# Autodesk Inventor assembly: ASSEMBLY_Y_axis_motor
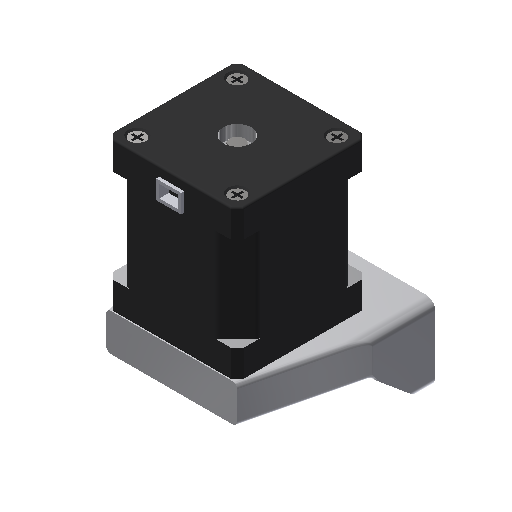
[picture p0: Inventor's stored thumbnail of the model, 512x512]
Saved by Autodesk Inventor 2026.1 (Build 301233000, 233)
## iProperties
Created: 2018-07-08
Part Number: ASSEMBLY_Y_axis_motor
Document SubType Name: Assembly
Designer: Andrzej
Author: Andrzej
## Documents named in this file (6)
- C:\Users\Andrzej\OneDrive\_DRIVE_SYNCH_FILES\__ BYTECHLAB PROJECTS\MLTDIS - SMD Parts Sorting Machine\MCAD\1_REV1\ASSEMBLY_XY_AXIS_REVA\ASSEMBLY_Y_axis_motor.iam
- C:\Users\Andrzej\OneDrive\_DRIVE_SYNCH_FILES\__ BYTECHLAB PROJECTS\MLTDIS - SMD Parts Sorting Machine\MCAD\1_REV1\ASSEMBLY_XY_AXIS_REVA\3DP_PLA_Nema_17_motor_mount.ipt
- C:\Users\Andrzej\OneDrive\_DRIVE_SYNCH_FILES\__ BYTECHLAB PROJECTS\MLTDIS - SMD Parts Sorting Machine\MCAD\1_REV1\__COTS_PARTS\COTS_GENERIC_NEMA_17_Stepper_motor.ipt
- C:\Users\Andrzej\OneDrive\_DRIVE_SYNCH_FILES\__ BYTECHLAB PROJECTS\MLTDIS - SMD Parts Sorting Machine\MCAD\1_REV1\__COTS_PARTS\COTS_GENERIC_GT2_20T_Pulley.ipt
- C:\Users\Andrzej\OneDrive\_DRIVE_SYNCH_FILES\__ BYTECHLAB PROJECTS\MLTDIS - SMD Parts Sorting Machine\MCAD\1_REV1\__CONTENT_CENTER_PARTS\en-US\DIN 125-2  A\DIN 125-2 - A 3,2A.ipt
- C:\Users\Andrzej\OneDrive\_DRIVE_SYNCH_FILES\__ BYTECHLAB PROJECTS\MLTDIS - SMD Parts Sorting Machine\MCAD\1_REV1\__CONTENT_CENTER_PARTS\en-US\ISO 7380-1\ISO 7380-1 - M3 x 20.ipt
## Components (11 placed, 5 different names)
1. 3DP_PLA_Nema_17_motor_mount:1 — Mate:1, Mate:2, Flush:1, Mate:4, Mate:5, Mate:6, Mate:7, Mate:8, Mate:9, Mate:10, Mate:11
2. COTS_GENERIC_NEMA_17_Stepper_motor:1 — Mate:1, Mate:2, Flush:1, Mate:3, Flush:2
3. COTS_GENERIC_GT2_20T_Pulley:1 — Mate:3, Flush:2
4. DIN 125-2 A A 3,2:1 — Mate:4, Mate:5, Insert:1
5. ISO 7380-1 M3 x 20:1 — Insert:1
6. DIN 125-2 A A 3,2:2 — Mate:6, Mate:7, Insert:2
7. DIN 125-2 A A 3,2:3 — Mate:8, Mate:9, Insert:3
8. DIN 125-2 A A 3,2:4 — Mate:10, Mate:11, Insert:4
9. ISO 7380-1 M3 x 20:2 — Insert:2
10. ISO 7380-1 M3 x 20:3 — Insert:3
11. ISO 7380-1 M3 x 20:4 — Insert:4
## Relationships (17: Mate 11, Insert 4, Flush 2)
- Mate:1: 3DP_PLA_Nema_17_motor_mount:1 ↔ COTS_GENERIC_NEMA_17_Stepper_motor:1
- Mate:2: 3DP_PLA_Nema_17_motor_mount:1 ↔ COTS_GENERIC_NEMA_17_Stepper_motor:1
- Flush:1: 3DP_PLA_Nema_17_motor_mount:1 ↔ COTS_GENERIC_NEMA_17_Stepper_motor:1
- Mate:3: COTS_GENERIC_NEMA_17_Stepper_motor:1 ↔ COTS_GENERIC_GT2_20T_Pulley:1
- Flush:2 (-1 mm): COTS_GENERIC_NEMA_17_Stepper_motor:1 ↔ COTS_GENERIC_GT2_20T_Pulley:1
- Mate:4: 3DP_PLA_Nema_17_motor_mount:1 ↔ DIN 125-2 A A 3,2:1
- Mate:5: 3DP_PLA_Nema_17_motor_mount:1 ↔ DIN 125-2 A A 3,2:1
- Mate:6: 3DP_PLA_Nema_17_motor_mount:1 ↔ DIN 125-2 A A 3,2:2
- Mate:7: 3DP_PLA_Nema_17_motor_mount:1 ↔ DIN 125-2 A A 3,2:2
- Mate:8: 3DP_PLA_Nema_17_motor_mount:1 ↔ DIN 125-2 A A 3,2:3
- Mate:9: 3DP_PLA_Nema_17_motor_mount:1 ↔ DIN 125-2 A A 3,2:3
- Mate:10: 3DP_PLA_Nema_17_motor_mount:1 ↔ DIN 125-2 A A 3,2:4
- Mate:11: 3DP_PLA_Nema_17_motor_mount:1 ↔ DIN 125-2 A A 3,2:4
- Insert:1: DIN 125-2 A A 3,2:1 ↔ ISO 7380-1 M3 x 20:1
- Insert:2: DIN 125-2 A A 3,2:2 ↔ ISO 7380-1 M3 x 20:2
- Insert:3: DIN 125-2 A A 3,2:3 ↔ ISO 7380-1 M3 x 20:3
- Insert:4: DIN 125-2 A A 3,2:4 ↔ ISO 7380-1 M3 x 20:4
